# Autodesk Inventor assembly: Robot Chassis - The actual one
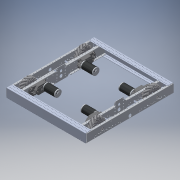
[picture p0: Inventor's stored thumbnail of the model, 180x180]
Saved by Autodesk Inventor 2017 (Build 210142000, 142)
## iProperties
Created: 2017-01-10
Part Number: Robot Chassis - The actual one
Document SubType Name: Assembly
Designer: Roksbot
Author: Roksbot
## Documents named in this file (5)
- C:\Users\Roksbot\Documents\Inventor\2017 Robot\Robot Chassis - The actual one.iam
- C:\Users\Roksbot\Documents\Inventor\2017 Robot\Short Build Volume.ipt
- C:\Users\Roksbot\Documents\Inventor\2017 Robot\Tall Build Volume.ipt
- C:\Users\Roksbot\Documents\Inventor\2017 Robot\Robot Chassis Half.iam
- C:\Users\Roksbot\Documents\Inventor\2017 Robot\End Sheet - 28.5.ipt
## Components (6 placed, 4 different names)
1. Short Build Volume:1 — Flush:5, Flush:6, Flush:7, Flush:9, Flush:14
2. Tall Build Volume:1 — Flush:5, Flush:6, Flush:7, Flush:12
3. Robot Chassis Half:1 [sub-assembly] — Flush:9, Flush:11, Mate:1, Flush:12, Flush:13, Insert:3
4. Robot Chassis Half:2 [sub-assembly] — Flush:11, Mate:1, Flush:13, Insert:1, Insert:4
5. End Sheet - 28.5:1 — Insert:3, Insert:4
6. End Sheet - 28.5:2 — Insert:1, Flush:14
## Relationships (12: Flush 8, Insert 3, Mate 1)
- Flush:5: Short Build Volume:1 ↔ Tall Build Volume:1
- Flush:6: Short Build Volume:1 ↔ Tall Build Volume:1
- Flush:7: Short Build Volume:1 ↔ Tall Build Volume:1
- Flush:9 (-38.1 mm): Short Build Volume:1 ↔ Robot Chassis Half:1
- Flush:11: Robot Chassis Half:1 ↔ Robot Chassis Half:2
- Mate:1 (723.9 mm): Robot Chassis Half:1 ↔ Robot Chassis Half:2
- Flush:12 (88.9 mm): Tall Build Volume:1 ↔ Robot Chassis Half:1
- Flush:13: Robot Chassis Half:1 ↔ Robot Chassis Half:2
- Insert:1: Robot Chassis Half:2 ↔ End Sheet - 28.5:2
- Flush:14 (-88.9 mm): Short Build Volume:1 ↔ End Sheet - 28.5:2
- Insert:3: Robot Chassis Half:1 ↔ End Sheet - 28.5:1
- Insert:4: Robot Chassis Half:2 ↔ End Sheet - 28.5:1
